# Autodesk Inventor assembly: Robot4
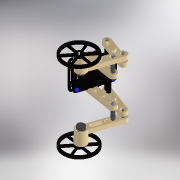
[picture p0: Inventor's stored thumbnail of the model, 180x180]
Saved by Autodesk Inventor 2021 (Build 250183000, 183)
## iProperties
Created: 2024-04-10
Part Number: Robot4
Document SubType Name: Assembly
Designer: Martin
Author: Martin
## Documents named in this file (18)
- C:\Users\ASUS\OneDrive - Universidad de Antioquia\2024-1\Robótica\Proyecto\CAD\op1\Robot4.iam
- C:\Users\ASUS\OneDrive - Universidad de Antioquia\2024-1\Robótica\Proyecto\CAD\op1\BaseEnsamble.iam
- C:\Users\ASUS\Documents\Inventor\Content Center Files\R2021\en-US\GB_T 276-94 60000-RS and LS\Bearing 61900-LS GB_T 276-94.ipt
- C:\Users\ASUS\Documents\Inventor\Content Center Files\R2021\en-US\AS 1111\AS 1111 - M8 x 90.ipt
- C:\Users\ASUS\Documents\Inventor\Content Center Files\R2021\en-US\ISO 1207(2)\ISO 1207 - M8 x 50.ipt
- C:\Users\ASUS\Documents\Inventor\Content Center Files\R2021\en-US\AS 1112 (2)\AS 1112 - M8  Type 5.ipt
- C:\Users\ASUS\OneDrive - Universidad de Antioquia\2024-1\Robótica\Proyecto\CAD\op1\EslabonCodoTrasero_MIR2.ipt
- C:\Users\ASUS\OneDrive - Universidad de Antioquia\2024-1\Robótica\Proyecto\CAD\op1\EslabonRodillaCadera_MIR2.ipt
- C:\Users\ASUS\OneDrive - Universidad de Antioquia\2024-1\Robótica\Proyecto\CAD\op1\EslabonRuedaRodilla_MIR2.ipt
- C:\Users\ASUS\OneDrive - Universidad de Antioquia\2024-1\Robótica\Proyecto\CAD\op1\Llana_MIR1.ipt
- C:\Users\ASUS\OneDrive - Universidad de Antioquia\2024-1\Robótica\Proyecto\CAD\37d-gearmotor-19-30-encoder_MIR2.ipt
- C:\Users\ASUS\OneDrive - Universidad de Antioquia\2024-1\Robótica\Proyecto\CAD\Resorte_MIR3.ipt
- C:\Users\ASUS\OneDrive - Universidad de Antioquia\2024-1\Robótica\Proyecto\CAD\op1\EslabonCodoTrasero_MIR2_MIR.ipt
- C:\Users\ASUS\OneDrive - Universidad de Antioquia\2024-1\Robótica\Proyecto\CAD\op1\EslabonRodillaCadera_MIR2_MIR.ipt
- C:\Users\ASUS\OneDrive - Universidad de Antioquia\2024-1\Robótica\Proyecto\CAD\op1\EslabonRuedaRodilla_MIR2_MIR.ipt
- C:\Users\ASUS\OneDrive - Universidad de Antioquia\2024-1\Robótica\Proyecto\CAD\op1\Llana_MIR1_MIR.ipt
- C:\Users\ASUS\OneDrive - Universidad de Antioquia\2024-1\Robótica\Proyecto\CAD\37d-gearmotor-19-30-encoder_MIR2_MIR.ipt
- C:\Users\ASUS\OneDrive - Universidad de Antioquia\2024-1\Robótica\Proyecto\CAD\Resorte_MIR3_MIR.ipt
## Components (36 placed, 17 different names)
1. BaseEnsamble:1 [sub-assembly] — Insert:1
2. AS 1112 (2) - Metric M8  Type 5:1 — Insert:1
3. EslabonCodoTrasero_MIR2:1 — Mate:33, Mate:34, Mate:46, Mate:47, Mate:56, Mate:57, Insert:4, Insert:5
4. EslabonRodillaCadera_MIR2:1 — Mate:35, Mate:36, Mate:42, Mate:43
5. EslabonRuedaRodilla_MIR2:1 — Mate:33, Mate:34, Mate:35, Mate:36, Mate:37, Mate:39, Mate:40, Mate:41, Mate:44, Mate:45, Mate:50, Mate:51, Mate:52, Mate:53, Mate:54, Mate:55, Flush:1
6. Llana_MIR1:1 — Mate:37, Mate:38
7. 37d-gearmotor-19-30-encoder_MIR2:1 — Mate:38, Mate:39, Mate:40
8. Resorte_MIR3:1 — Mate:41
9. Rolling bearing GB/T 276-1994 Type 60000-RS and LS 61900-LS:6 — Mate:42, Mate:43
10. Rolling bearing GB/T 276-1994 Type 60000-RS and LS 61900-LS:7 — Mate:44, Mate:45
11. Rolling bearing GB/T 276-1994 Type 60000-RS and LS 61900-LS:8 — Mate:46, Mate:47, Mate:58
12. Rolling bearing GB/T 276-1994 Type 60000-RS and LS 61900-LS:9
13. Rolling bearing GB/T 276-1994 Type 60000-RS and LS 61900-LS:10 — Mate:50, Mate:51
14. AS 1111 - Metric M8 x 90:3 — Mate:52, Mate:53, Mate:60
15. ISO 1207 M8 x 50:2 — Mate:54, Mate:55, Mate:59
16. AS 1111 - Metric M8 x 90:4 — Mate:56, Mate:57
17. AS 1112 (2) - Metric M8  Type 5:6
18. AS 1112 (2) - Metric M8  Type 5:7 — Mate:58, Mate:59
19. AS 1112 (2) - Metric M8  Type 5:8 — Insert:4
20. AS 1112 (2) - Metric M8  Type 5:9 — Insert:5
21. AS 1112 (2) - Metric M8  Type 5:10 — Mate:60
22. EslabonCodoTrasero_MIR2_MIR:1 — Mate:63, Mate:64, Mate:74, Mate:75, Insert:6, Mate:79
23. EslabonRodillaCadera_MIR2_MIR:1 — Mate:61, Mate:62, Mate:77
24. EslabonRuedaRodilla_MIR2_MIR:1 — Mate:61, Mate:62, Mate:63, Mate:64, Mate:65, Mate:66, Mate:67, Mate:69, Mate:70, Mate:71, Mate:72, Mate:73, Mate:78
25. Llana_MIR1_MIR:1 — Mate:65, Mate:68
26. 37d-gearmotor-19-30-encoder_MIR2_MIR:1 — Mate:66, Mate:67, Mate:68
27. Resorte_MIR3_MIR:1 — Mate:69
28. AS 1111 - Metric M8 x 90:5 — Mate:70, Mate:71, Mate:76
29. ISO 1207 M8 x 50:3 — Mate:72, Mate:73
30. AS 1111 - Metric M8 x 90:6 — Mate:74, Mate:75
31. AS 1112 (2) - Metric M8  Type 5:11 — Insert:6
32. AS 1112 (2) - Metric M8  Type 5:12 — Mate:76
33. Rolling bearing GB/T 276-1994 Type 60000-RS and LS 61900-LS:11 — Flush:1
34. Rolling bearing GB/T 276-1994 Type 60000-RS and LS 61900-LS:12 — Mate:77
35. Rolling bearing GB/T 276-1994 Type 60000-RS and LS 61900-LS:13 — Mate:78
36. Rolling bearing GB/T 276-1994 Type 60000-RS and LS 61900-LS:14 — Mate:79
## Relationships (50: Mate 45, Insert 4, Flush 1)
- Insert:1: BaseEnsamble:1 ↔ AS 1112 (2) - Metric M8  Type 5:1
- Mate:33 (10 mm): EslabonCodoTrasero_MIR2:1 ↔ EslabonRuedaRodilla_MIR2:1
- Mate:34: EslabonCodoTrasero_MIR2:1 ↔ EslabonRuedaRodilla_MIR2:1
- Mate:35 (46 mm): EslabonRodillaCadera_MIR2:1 ↔ EslabonRuedaRodilla_MIR2:1
- Mate:36: EslabonRodillaCadera_MIR2:1 ↔ EslabonRuedaRodilla_MIR2:1
- Mate:37 (2 mm): EslabonRuedaRodilla_MIR2:1 ↔ Llana_MIR1:1
- Mate:38: Llana_MIR1:1 ↔ 37d-gearmotor-19-30-encoder_MIR2:1
- Mate:39: EslabonRuedaRodilla_MIR2:1 ↔ 37d-gearmotor-19-30-encoder_MIR2:1
- Mate:40: EslabonRuedaRodilla_MIR2:1 ↔ 37d-gearmotor-19-30-encoder_MIR2:1
- Mate:41: EslabonRuedaRodilla_MIR2:1 ↔ Resorte_MIR3:1
- Mate:42: EslabonRodillaCadera_MIR2:1 ↔ Rolling bearing GB/T 276-1994 Type 60000-RS and LS 61900-LS:6
- Mate:43: EslabonRodillaCadera_MIR2:1 ↔ Rolling bearing GB/T 276-1994 Type 60000-RS and LS 61900-LS:6
- Mate:44: EslabonRuedaRodilla_MIR2:1 ↔ Rolling bearing GB/T 276-1994 Type 60000-RS and LS 61900-LS:7
- Mate:45: EslabonRuedaRodilla_MIR2:1 ↔ Rolling bearing GB/T 276-1994 Type 60000-RS and LS 61900-LS:7
- Mate:46: EslabonCodoTrasero_MIR2:1 ↔ Rolling bearing GB/T 276-1994 Type 60000-RS and LS 61900-LS:8
- Mate:47: EslabonCodoTrasero_MIR2:1 ↔ Rolling bearing GB/T 276-1994 Type 60000-RS and LS 61900-LS:8
- Mate:50: EslabonRuedaRodilla_MIR2:1 ↔ Rolling bearing GB/T 276-1994 Type 60000-RS and LS 61900-LS:10
- Mate:51: EslabonRuedaRodilla_MIR2:1 ↔ Rolling bearing GB/T 276-1994 Type 60000-RS and LS 61900-LS:10
- Mate:52: EslabonRuedaRodilla_MIR2:1 ↔ AS 1111 - Metric M8 x 90:3
- Mate:53: EslabonRuedaRodilla_MIR2:1 ↔ AS 1111 - Metric M8 x 90:3
- Mate:54: EslabonRuedaRodilla_MIR2:1 ↔ ISO 1207 M8 x 50:2
- Mate:55: EslabonRuedaRodilla_MIR2:1 ↔ ISO 1207 M8 x 50:2
- Mate:56: EslabonCodoTrasero_MIR2:1 ↔ AS 1111 - Metric M8 x 90:4
- Mate:57: EslabonCodoTrasero_MIR2:1 ↔ AS 1111 - Metric M8 x 90:4
- Mate:58: Rolling bearing GB/T 276-1994 Type 60000-RS and LS 61900-LS:8 ↔ AS 1112 (2) - Metric M8  Type 5:7
- Mate:59: ISO 1207 M8 x 50:2 ↔ AS 1112 (2) - Metric M8  Type 5:7
- Insert:4: EslabonCodoTrasero_MIR2:1 ↔ AS 1112 (2) - Metric M8  Type 5:8
- Insert:5: EslabonCodoTrasero_MIR2:1 ↔ AS 1112 (2) - Metric M8  Type 5:9
- Mate:60: AS 1111 - Metric M8 x 90:3 ↔ AS 1112 (2) - Metric M8  Type 5:10
- Mate:61: EslabonRodillaCadera_MIR2_MIR:1 ↔ EslabonRuedaRodilla_MIR2_MIR:1
- Mate:62 (46 mm): EslabonRodillaCadera_MIR2_MIR:1 ↔ EslabonRuedaRodilla_MIR2_MIR:1
- Mate:63: EslabonCodoTrasero_MIR2_MIR:1 ↔ EslabonRuedaRodilla_MIR2_MIR:1
- Mate:64 (10 mm): EslabonCodoTrasero_MIR2_MIR:1 ↔ EslabonRuedaRodilla_MIR2_MIR:1
- Mate:65 (2 mm): EslabonRuedaRodilla_MIR2_MIR:1 ↔ Llana_MIR1_MIR:1
- Mate:66: EslabonRuedaRodilla_MIR2_MIR:1 ↔ 37d-gearmotor-19-30-encoder_MIR2_MIR:1
- Mate:67: EslabonRuedaRodilla_MIR2_MIR:1 ↔ 37d-gearmotor-19-30-encoder_MIR2_MIR:1
- Mate:68: Llana_MIR1_MIR:1 ↔ 37d-gearmotor-19-30-encoder_MIR2_MIR:1
- Mate:69: EslabonRuedaRodilla_MIR2_MIR:1 ↔ Resorte_MIR3_MIR:1
- Mate:70: EslabonRuedaRodilla_MIR2_MIR:1 ↔ AS 1111 - Metric M8 x 90:5
- Mate:71: EslabonRuedaRodilla_MIR2_MIR:1 ↔ AS 1111 - Metric M8 x 90:5
- Mate:72: EslabonRuedaRodilla_MIR2_MIR:1 ↔ ISO 1207 M8 x 50:3
- Mate:73: EslabonRuedaRodilla_MIR2_MIR:1 ↔ ISO 1207 M8 x 50:3
- Mate:74: EslabonCodoTrasero_MIR2_MIR:1 ↔ AS 1111 - Metric M8 x 90:6
- Mate:75: EslabonCodoTrasero_MIR2_MIR:1 ↔ AS 1111 - Metric M8 x 90:6
- Insert:6: EslabonCodoTrasero_MIR2_MIR:1 ↔ AS 1112 (2) - Metric M8  Type 5:11
- Mate:76: AS 1111 - Metric M8 x 90:5 ↔ AS 1112 (2) - Metric M8  Type 5:12
- Flush:1: EslabonRuedaRodilla_MIR2:1 ↔ Rolling bearing GB/T 276-1994 Type 60000-RS and LS 61900-LS:11
- Mate:77: EslabonRodillaCadera_MIR2_MIR:1 ↔ Rolling bearing GB/T 276-1994 Type 60000-RS and LS 61900-LS:12
- Mate:78: EslabonRuedaRodilla_MIR2_MIR:1 ↔ Rolling bearing GB/T 276-1994 Type 60000-RS and LS 61900-LS:13
- Mate:79: EslabonCodoTrasero_MIR2_MIR:1 ↔ Rolling bearing GB/T 276-1994 Type 60000-RS and LS 61900-LS:14
